# Autodesk Inventor assembly: mobile
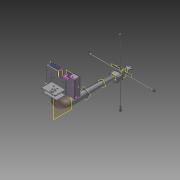
[picture p0: Inventor's stored thumbnail of the model, 180x180]
Saved by Autodesk Inventor 2014 SP2 (Build 180247200, 247)
## iProperties
Created: 2017-08-03
Part Number: mobile
Document SubType Name: Assembly
Designer: hide
Author: hide
## Documents named in this file (16)
- C:\Users\hide\src\github.com\stem-dad\diy-baby-crib-mobile\models\mobile.iam
- C:\Users\hide\src\github.com\stem-dad\diy-baby-crib-mobile\models\pole-bottom.ipt
- C:\Users\hide\src\github.com\stem-dad\diy-baby-crib-mobile\models\pole-center.ipt
- C:\Users\hide\src\github.com\stem-dad\diy-baby-crib-mobile\models\pole-top.ipt
- C:\Users\hide\src\github.com\stem-dad\diy-baby-crib-mobile\models\stick-holder-top2.ipt
- C:\Users\hide\src\github.com\stem-dad\diy-baby-crib-mobile\models\top-star.ipt
- C:\Users\hide\src\github.com\stem-dad\diy-baby-crib-mobile\models\motor-holder.ipt
- C:\Users\hide\src\github.com\stem-dad\diy-baby-crib-mobile\models\pole-corner.ipt
- C:\Users\hide\src\github.com\stem-dad\diy-baby-crib-mobile\models\bed-stopper.ipt
- C:\Users\hide\src\github.com\stem-dad\diy-baby-crib-mobile\models\arduino-holder.ipt
- C:\Users\hide\src\github.com\stem-dad\diy-baby-crib-mobile\models\arduino-holder-cover.ipt
- C:\Users\hide\src\github.com\stem-dad\diy-baby-crib-mobile\models\raspi-holder.ipt
- C:\Users\hide\src\github.com\stem-dad\diy-baby-crib-mobile\models\raspi-holder-top.ipt
- C:\Users\hide\src\github.com\stem-dad\diy-baby-crib-mobile\models\raspi-holder-top-speaker.ipt
- C:\Users\hide\src\github.com\stem-dad\diy-baby-crib-mobile\models\stick.ipt
- C:\Users\hide\src\github.com\stem-dad\diy-baby-crib-mobile\models\stick-cap.ipt
## Components (19 placed, 15 different names)
1. pole-bottom:1 — メイト:1, メイト:2, メイト:3, メイト:14, メイト:15, メイト:19
2. pole-center:1 — メイト:1, メイト:2, メイト:3, メイト:4, メイト:5, メイト:6
3. pole-top:1 — メイト:4, メイト:5, メイト:6, メイト:31, フラッシュ:3, メイト:32, 角度:5
4. stick-holder-top2:1 — メイト:9, メイト:10, 角度:1, メイト:33, メイト:34, メイト:43, メイト:44, フラッシュ:7, フラッシュ:8, 角度:3, 角度:4
5. top-star:1 — メイト:9, メイト:10, 角度:1, 角度:7
6. motor-holder:1 — メイト:31, フラッシュ:3, メイト:32, メイト:33, メイト:34, 角度:6
7. pole-corner:1 — メイト:14, メイト:15, メイト:17, メイト:18, メイト:19, メイト:20
8. bed-stopper:1 — メイト:17, メイト:18, メイト:20, メイト:22, メイト:23, メイト:24, メイト:40, 角度:2, メイト:41
9. arduino-holder:1 — メイト:22, メイト:23, メイト:24, メイト:30, フラッシュ:1, フラッシュ:2, メイト:42, 角度:7
10. arduino-holder-cover:1 — メイト:30, フラッシュ:1, フラッシュ:2
11. raspi-holder:1 — メイト:38, フラッシュ:4, フラッシュ:5, メイト:40, 角度:2, メイト:41, フラッシュ:6
12. raspi-holder-top:1 — メイト:35, メイト:36, メイト:37, メイト:38, フラッシュ:4, フラッシュ:5
13. raspi-holder-top-speaker:1 — メイト:35, メイト:36, メイト:37
14. stick:1 — メイト:43, フラッシュ:8, メイト:47, メイト:48, メイト:49, メイト:50
15. stick:2 — メイト:44, フラッシュ:7, メイト:45, メイト:46, メイト:51, メイト:52
16. stick-cap:1 — メイト:45, メイト:46, 角度:3
17. stick-cap:2 — メイト:49, メイト:50, 角度:5
18. stick-cap:3 — メイト:47, 角度:4, メイト:48
19. stick-cap:4 — メイト:51, メイト:52, 角度:6
## Relationships (54: Mate 39, Flush 8, Angle 7)
- メイト:1 [Mate]: pole-bottom:1 ↔ pole-center:1
- メイト:2 [Mate]: pole-bottom:1 ↔ pole-center:1
- メイト:3 [Mate]: pole-bottom:1 ↔ pole-center:1
- メイト:4 [Mate]: pole-center:1 ↔ pole-top:1
- メイト:5 [Mate]: pole-center:1 ↔ pole-top:1
- メイト:6 [Mate]: pole-center:1 ↔ pole-top:1
- メイト:9 [Mate]: stick-holder-top2:1 ↔ top-star:1
- メイト:10 [Mate]: stick-holder-top2:1 ↔ top-star:1
- 角度:1 [Angle] (0 deg): stick-holder-top2:1 ↔ top-star:1
- メイト:14 [Mate]: pole-bottom:1 ↔ pole-corner:1
- メイト:15 [Mate]: pole-bottom:1 ↔ pole-corner:1
- メイト:17 [Mate]: pole-corner:1 ↔ bed-stopper:1
- メイト:18 [Mate]: pole-corner:1 ↔ bed-stopper:1
- メイト:19 [Mate]: pole-bottom:1 ↔ pole-corner:1
- メイト:20 [Mate]: pole-corner:1 ↔ bed-stopper:1
- メイト:22 [Mate]: bed-stopper:1 ↔ arduino-holder:1
- メイト:23 [Mate]: bed-stopper:1 ↔ arduino-holder:1
- メイト:24 [Mate]: bed-stopper:1 ↔ arduino-holder:1
- メイト:30 [Mate]: arduino-holder:1 ↔ arduino-holder-cover:1
- フラッシュ:1 [Flush]: arduino-holder:1 ↔ arduino-holder-cover:1
- フラッシュ:2 [Flush]: arduino-holder:1 ↔ arduino-holder-cover:1
- メイト:31 [Mate]: pole-top:1 ↔ motor-holder:1
- フラッシュ:3 [Flush]: pole-top:1 ↔ motor-holder:1
- メイト:32 [Mate]: pole-top:1 ↔ motor-holder:1
- メイト:33 [Mate]: stick-holder-top2:1 ↔ motor-holder:1
- メイト:34 [Mate]: stick-holder-top2:1 ↔ motor-holder:1
- メイト:35 [Mate]: raspi-holder-top:1 ↔ raspi-holder-top-speaker:1
- メイト:36 [Mate]: raspi-holder-top:1 ↔ raspi-holder-top-speaker:1
- メイト:37 [Mate]: raspi-holder-top:1 ↔ raspi-holder-top-speaker:1
- メイト:38 [Mate]: raspi-holder:1 ↔ raspi-holder-top:1
- フラッシュ:4 [Flush]: raspi-holder:1 ↔ raspi-holder-top:1
- フラッシュ:5 [Flush]: raspi-holder:1 ↔ raspi-holder-top:1
- メイト:40 [Mate]: bed-stopper:1 ↔ raspi-holder:1
- 角度:2 [Angle] (0 deg): bed-stopper:1 ↔ raspi-holder:1
- メイト:41 [Mate]: bed-stopper:1 ↔ raspi-holder:1
- フラッシュ:6 [Flush]: raspi-holder:1
- メイト:42 [Mate]: arduino-holder:1
- メイト:43 [Mate]: stick-holder-top2:1 ↔ stick:1
- メイト:44 [Mate]: stick-holder-top2:1 ↔ stick:2
- フラッシュ:7 [Flush] (157 mm): stick-holder-top2:1 ↔ stick:2
- フラッシュ:8 [Flush] (157 mm): stick-holder-top2:1 ↔ stick:1
- メイト:45 [Mate]: stick:2 ↔ stick-cap:1
- メイト:46 [Mate] (-10 mm): stick:2 ↔ stick-cap:1
- 角度:3 [Angle] (90 deg): stick-holder-top2:1 ↔ stick-cap:1
- メイト:47 [Mate]: stick:1 ↔ stick-cap:3
- 角度:4 [Angle] (90 deg): stick-holder-top2:1 ↔ stick-cap:3
- メイト:48 [Mate] (-10 mm): stick:1 ↔ stick-cap:3
- メイト:49 [Mate]: stick:1 ↔ stick-cap:2
- メイト:50 [Mate] (-10 mm): stick:1 ↔ stick-cap:2
- 角度:5 [Angle] (90 deg): pole-top:1 ↔ stick-cap:2
- メイト:51 [Mate]: stick:2 ↔ stick-cap:4
- メイト:52 [Mate] (-10 mm): stick:2 ↔ stick-cap:4
- 角度:6 [Angle] (90 deg): motor-holder:1 ↔ stick-cap:4
- 角度:7 [Angle] (180 deg): top-star:1 ↔ arduino-holder:1
